# Autodesk Inventor assembly: Botkit-Hubs
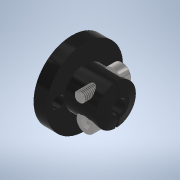
[picture p0: Inventor's stored thumbnail of the model, 180x180]
Saved by Autodesk Inventor 2022 (Build 260153000, 153)
## iProperties
Created: 2022-07-25
Part Number: Botkit-Hubs
Document SubType Name: Assembly
Designer: Nathan Cai
Author: Nathan Cai
## Documents named in this file (3)
- C:\Users\Nathan Cai\Documents\Inventor\Asorted Parts\Botkit-Hubs.iam
- C:\Users\Nathan Cai\Documents\Inventor\Asorted Parts\Hub.ipt
- C:\Users\Nathan Cai\Documents\Inventor\Content Center Files\R2022\en-US\ISO 4762(2)\ISO 4762 - M3 x 10ISO.ipt
## Components (3 placed, 2 different names)
1. Hub:1 — Mate:1, Mate:2, Mate:3, Mate:4
2. ISO 4762 M3 x 10:2 — Mate:1, Mate:2
3. ISO 4762 M3 x 10:3 — Mate:3, Mate:4
## Relationships (4: Mate 4)
- Mate:1: Hub:1 ↔ ISO 4762 M3 x 10:2
- Mate:2: Hub:1 ↔ ISO 4762 M3 x 10:2
- Mate:3: Hub:1 ↔ ISO 4762 M3 x 10:3
- Mate:4: Hub:1 ↔ ISO 4762 M3 x 10:3
